# Autodesk Inventor assembly: 305-04
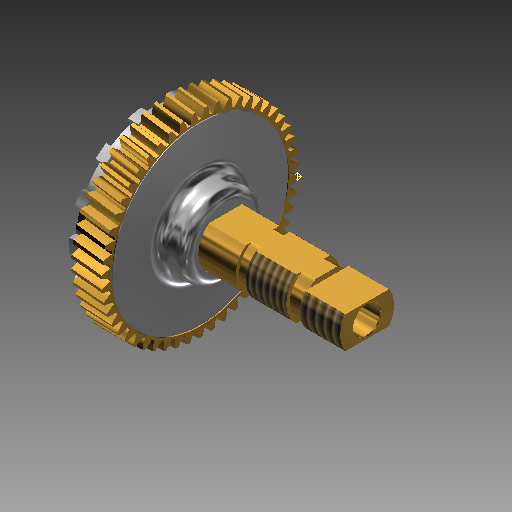
[picture p0: Inventor's stored thumbnail of the model, 512x512]
Saved by Autodesk Inventor 2019 (Build 230136000, 136)
## iProperties
Company: Autodesk Inc.
Created: 2012-01-27
Part Number: 305-04
Document SubType Name: Assembly
Designer: Autodesk Inc.
Mass: 35.6728 g
Surface Area: 70.3136 cm^2
Volume: 4.33332 cm^3
Density: 8.2322 g/cm^3
Author: Inventor
## Documents named in this file (7)
- C:\TEMP\Fishing Rod\Workspaces\Crankshaft Assembly.iam
- C:\TEMP\Fishing Rod\Workspaces\Crankshaft.ipt
- C:\TEMP\Fishing Rod\Workspaces\Drag Sprocket Pin.ipt
- C:\TEMP\Fishing Rod\Workspaces\Drag Sprocket.ipt
- C:\TEMP\Fishing Rod\Workspaces\Drive Gear Offset Spacer B.ipt
- C:\TEMP\Fishing Rod\Workspaces\Main Drive Gear.iam
- C:\TEMP\Fishing Rod\Workspaces\Drive Gear Offset Spacer A.ipt
## Components (7 placed, 6 different names)
1. Crankshaft:1 — Insert:3, Angle:1, Angle:2, Angle:3, Mate:2, Mate:3
2. Drag Sprocket Pin:1 — Insert:1
3. Drag Sprocket:1 — Insert:1, Insert:2, Insert:3, Angle:1, Insert:4
4. Drag Sprocket Pin:2 — Insert:2
5. Drive Gear Offset Spacer B:1 — Insert:4, Angle:2, Mate:4
6. Main Drive Gear:1 [sub-assembly] — Mate:1, Mate:3, Mate:4, Mate:5
7. Drive Gear Offset Spacer A:1 — Angle:3, Mate:2, Mate:5
## Relationships (12: Mate 5, Insert 4, Angle 3)
- Insert:1: Drag Sprocket Pin:1 ↔ Drag Sprocket:1
- Insert:2: Drag Sprocket:1 ↔ Drag Sprocket Pin:2
- Insert:3: Crankshaft:1 ↔ Drag Sprocket:1
- Angle:1 (0 deg): Crankshaft:1 ↔ Drag Sprocket:1
- Insert:4: Drag Sprocket:1 ↔ Drive Gear Offset Spacer B:1
- Angle:2 (0 deg): Crankshaft:1 ↔ Drive Gear Offset Spacer B:1
- Angle:3 (0 deg): Crankshaft:1 ↔ Drive Gear Offset Spacer A:1
- Mate:1: Main Drive Gear:1
- Mate:2: Crankshaft:1 ↔ Drive Gear Offset Spacer A:1
- Mate:3: Crankshaft:1 ↔ Main Drive Gear:1
- Mate:4: Drive Gear Offset Spacer B:1 ↔ Main Drive Gear:1
- Mate:5: Main Drive Gear:1 ↔ Drive Gear Offset Spacer A:1
